# Autodesk Inventor assembly: Tattu 850mah 4S
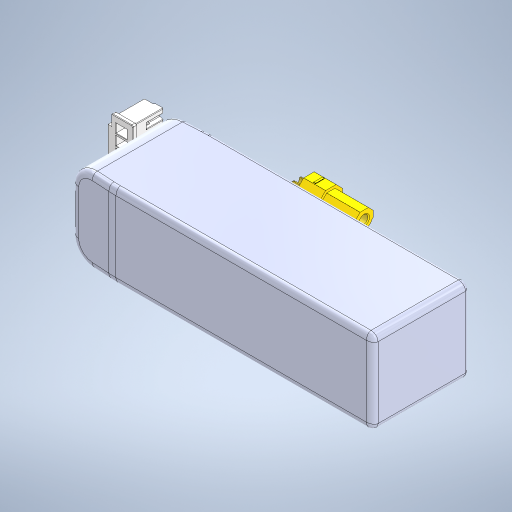
[picture p0: Inventor's stored thumbnail of the model, 512x512]
Saved by Autodesk Inventor 2023.4 (Build 274418000, 418)
## iProperties
Created: 2022-12-23
Part Number: Tattu 850mah 4S
Document SubType Name: Assembly
Designer: Nathan Cai
Mass: 104 g
Surface Area: 183.891 cm^2
Volume: 2.44269 cm^3
Author: Nathan Cai
## Documents named in this file (4)
- E:\Documents\Inventor\Shin Impact V1.0\Tattu 4S 850mah\Tattu 850mah 4S.iam
- E:\Documents\Inventor\Shin Impact V1.0\Tattu 4S 850mah\FUNDA 13.ipt
- E:\Documents\Inventor\Shin Impact V1.0\Tattu 4S 850mah\JST XHP-4.ipt
- E:\Documents\Inventor\Shin Impact V1.0\Tattu 4S 850mah\XdT30male.ipt
## Components (3 placed, 3 different names)
1. FUNDA 13:1 — Flush:2, Mate:2, Flush:3, Flush:4, Mate:3
2. JST XHP-4:1 — Flush:2, Mate:2, Flush:3
3. XdT30male:1 — Flush:4, Mate:3
## Relationships (5: Flush 3, Mate 2)
- Flush:2: FUNDA 13:1 ↔ JST XHP-4:1
- Mate:2: FUNDA 13:1 ↔ JST XHP-4:1
- Flush:3: FUNDA 13:1 ↔ JST XHP-4:1
- Flush:4: FUNDA 13:1 ↔ XdT30male:1
- Mate:3: FUNDA 13:1 ↔ XdT30male:1
